# Autodesk Inventor assembly: HF-Kabelführung-Back-Assembly
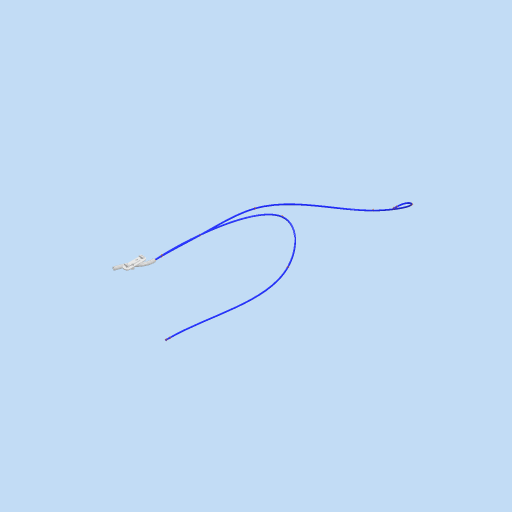
[picture p0: Inventor's stored thumbnail of the model, 512x512]
Saved by Autodesk Inventor 2023.2 (Build 272271000, 271)
## iProperties
Created: 2024-02-09
Part Number: HF-Kabelführung-Back-Assembly
Document SubType Name: Assembly
Designer: Nils Bade
Author: Nils Bade
## Documents named in this file (8)
- C:\Users\nilsb\Documents\Inventor\Projektarbeit-Bade\RatRig_Bade\HF-Kabelführung Measurement Chamber\HF-Kabelführung-Back-Assembly.iam
- C:\Users\nilsb\Documents\Inventor\Projektarbeit-Bade\RatRig_Bade\HF-Kabelführung Measurement Chamber\HF-Kabeldurchführung-BackPanel-Base.ipt
- C:\Users\nilsb\Documents\Inventor\Projektarbeit-Bade\RatRig_Bade\HF-Kabelführung Measurement Chamber\HF-Kabeldurchführung-BackPanel-Deckel.ipt
- C:\Users\nilsb\Documents\Inventor\Projektarbeit-Bade\Schrauben\Cap Head Screw M4x8 - DIN912.ipt
- C:\Users\nilsb\Documents\Inventor\Projektarbeit-Bade\RatRig_Standards\Hex Nut - M4 DIN934.ipt
- C:\Users\nilsb\Documents\Inventor\Projektarbeit-Bade\Schrauben\Cap Head Screw M6x12 v2.ipt
- C:\Users\nilsb\Documents\Inventor\Projektarbeit-Bade\RatRig_modified\T-NUT - DropIn 4040 SERIES - M6.ipt
- C:\Users\nilsb\Documents\Inventor\Projektarbeit-Bade\RatRig_Bade\HF-Kabelführung Measurement Chamber\HF-Kabelführung-V1-BackPlane-Kabellängen.iam
## Components (11 placed, 7 different names)
1. HF-Kabeldurchführung-BackPanel-Base:1 — Passend:1, Passend:2, Passend:3, Winkel:1, Winkel:2, Passend:10, Passend:11, Passend:12, Passend:13, Passend:14, Passend:15, Passend:16, Passend:17, Winkel:3, Winkel:4, Passend:18, Passend:19
2. HF-Kabeldurchführung-BackPanel-Deckel:1 — Passend:1, Passend:2, Passend:3, Passend:4, Passend:5, Passend:6, Passend:7, Passend:20
3. Cap Head Screw M4x8 - DIN912:1 — Passend:4, Passend:5, Passend:8
4. Cap Head Screw M4x8 - DIN912:2 — Passend:6, Passend:7, Passend:9
5. Hex Nut - M4 DIN934:1 — Passend:8, Winkel:1, Passend:10
6. Hex Nut - M4 DIN934:2 — Passend:9, Winkel:2, Passend:11
7. Cap Head Screw M6x12 v2:1 — Passend:12, Passend:14
8. Cap Head Screw M6x12 v2:2 — Passend:13, Passend:15
9. T-NUT - DROP IN TYPE FOR 40 SERIES - M6:1 — Passend:16, Winkel:3, Passend:18
10. T-NUT - DROP IN TYPE FOR 40 SERIES - M6:2 — Passend:17, Winkel:4, Passend:19
11. HF-Kabelführung-V1-BackPlane-Kabellängen:1 [sub-assembly] — Winkel:5, Winkel:6, Winkel:7, Passend:21
## Relationships (28: Mate 21, Angle 7)
- Passend:1 [Mate]: HF-Kabeldurchführung-BackPanel-Base:1 ↔ HF-Kabeldurchführung-BackPanel-Deckel:1
- Passend:2 [Mate]: HF-Kabeldurchführung-BackPanel-Base:1 ↔ HF-Kabeldurchführung-BackPanel-Deckel:1
- Passend:3 [Mate]: HF-Kabeldurchführung-BackPanel-Base:1 ↔ HF-Kabeldurchführung-BackPanel-Deckel:1
- Passend:4 [Mate]: HF-Kabeldurchführung-BackPanel-Deckel:1 ↔ Cap Head Screw M4x8 - DIN912:1
- Passend:5 [Mate]: HF-Kabeldurchführung-BackPanel-Deckel:1 ↔ Cap Head Screw M4x8 - DIN912:1
- Passend:6 [Mate]: HF-Kabeldurchführung-BackPanel-Deckel:1 ↔ Cap Head Screw M4x8 - DIN912:2
- Passend:7 [Mate]: HF-Kabeldurchführung-BackPanel-Deckel:1 ↔ Cap Head Screw M4x8 - DIN912:2
- Passend:8 [Mate]: Cap Head Screw M4x8 - DIN912:1 ↔ Hex Nut - M4 DIN934:1
- Passend:9 [Mate]: Cap Head Screw M4x8 - DIN912:2 ↔ Hex Nut - M4 DIN934:2
- Winkel:1 [Angle] (0 deg): HF-Kabeldurchführung-BackPanel-Base:1 ↔ Hex Nut - M4 DIN934:1
- Winkel:2 [Angle] (0 deg): HF-Kabeldurchführung-BackPanel-Base:1 ↔ Hex Nut - M4 DIN934:2
- Passend:10 [Mate]: HF-Kabeldurchführung-BackPanel-Base:1 ↔ Hex Nut - M4 DIN934:1
- Passend:11 [Mate]: HF-Kabeldurchführung-BackPanel-Base:1 ↔ Hex Nut - M4 DIN934:2
- Passend:12 [Mate]: HF-Kabeldurchführung-BackPanel-Base:1 ↔ Cap Head Screw M6x12 v2:1
- Passend:13 [Mate]: HF-Kabeldurchführung-BackPanel-Base:1 ↔ Cap Head Screw M6x12 v2:2
- Passend:14 [Mate]: HF-Kabeldurchführung-BackPanel-Base:1 ↔ Cap Head Screw M6x12 v2:1
- Passend:15 [Mate]: HF-Kabeldurchführung-BackPanel-Base:1 ↔ Cap Head Screw M6x12 v2:2
- Passend:16 [Mate]: HF-Kabeldurchführung-BackPanel-Base:1 ↔ T-NUT - DROP IN TYPE FOR 40 SERIES - M6:1
- Passend:17 [Mate]: HF-Kabeldurchführung-BackPanel-Base:1 ↔ T-NUT - DROP IN TYPE FOR 40 SERIES - M6:2
- Winkel:3 [Angle] (0 deg): HF-Kabeldurchführung-BackPanel-Base:1 ↔ T-NUT - DROP IN TYPE FOR 40 SERIES - M6:1
- Winkel:4 [Angle] (0 deg): HF-Kabeldurchführung-BackPanel-Base:1 ↔ T-NUT - DROP IN TYPE FOR 40 SERIES - M6:2
- Passend:18 [Mate] (4.5 mm): HF-Kabeldurchführung-BackPanel-Base:1 ↔ T-NUT - DROP IN TYPE FOR 40 SERIES - M6:1
- Passend:19 [Mate] (4.5 mm): HF-Kabeldurchführung-BackPanel-Base:1 ↔ T-NUT - DROP IN TYPE FOR 40 SERIES - M6:2
- Passend:20 [Mate]: HF-Kabeldurchführung-BackPanel-Deckel:1
- Winkel:5 [Angle] (0 deg): HF-Kabelführung-V1-BackPlane-Kabellängen:1
- Winkel:6 [Angle] (0 deg): HF-Kabelführung-V1-BackPlane-Kabellängen:1
- Winkel:7 [Angle] (0 deg): HF-Kabelführung-V1-BackPlane-Kabellängen:1
- Passend:21 [Mate]: HF-Kabelführung-V1-BackPlane-Kabellängen:1
